# Autodesk Inventor assembly: TR1 Actuator
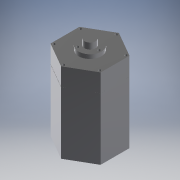
[picture p0: Inventor's stored thumbnail of the model, 180x180]
Saved by Autodesk Inventor 2017 (Build 210142000, 142)
## iProperties
Created: 2018-10-09
Part Number: TR1 Actuator
Document SubType Name: Assembly
Designer: Zach
Author: Zach
## Documents named in this file (15)
- C:\Users\Dell\Documents\GitHub\tr2\Arm Actuator\Arm Actuator.iam
- C:\Users\Dell\Documents\GitHub\tr2\Arm Actuator\TA01.ipt
- C:\Users\Dell\Documents\GitHub\tr2\Arm Actuator\TA02.ipt
- C:\Users\Dell\Documents\GitHub\tr2\Arm Actuator\Arm Actuator\Design Accelerator\Spur Gears2.iam
- C:\Users\Dell\Documents\GitHub\tr2\Arm Actuator\Arm Actuator\Design Accelerator\Spur Gears3.iam
- C:\Users\Dell\Documents\GitHub\tr2\Arm Actuator\EMS22XXX-D28-LSX.ipt
- C:\Users\Dell\Documents\GitHub\tr2\Arm Actuator\12RPM Gear Motor.ipt
- C:\Users\Dell\Documents\GitHub\tr2\Arm Actuator\Slip Ring.ipt
- C:\Users\Dell\Documents\GitHub\tr2\Arm Actuator\TA06.ipt
- C:\Users\Dell\Documents\GitHub\tr2\Arm Actuator\6mm Mounting Hub, thin.ipt
- C:\Users\Dell\Documents\GitHub\tr2\Arm Actuator\Steel Tubing.ipt
- C:\Users\Dell\Documents\GitHub\tr2\Arm Actuator\Flange Bearing.ipt
- C:\Users\Dell\Documents\GitHub\tr2\Arm Actuator\Shaft Collar.ipt
- C:\Users\Dell\Documents\GitHub\tr2\Arm Actuator\Arm Actuator\Design Accelerator\Spur Gear13.ipt
- C:\Users\Dell\Documents\GitHub\tr2\Arm Actuator\6mm Mounting Hub, thick.ipt
## Components (16 placed, 13 different names)
1. TA01:1 — Mate:28, Mate:29, Mate:30
2. TA02:1 — Mate:2, Angle:1, Mate:21, Mate:22, Mate:24, Mate:28, Mate:29, Mate:30, Mate:40, Mate:46, Mate:56, Flush:1, Mate:74, Mate:75, Mate:85, Mate:87, Mate:90, Mate:91
3. TA06:1 — Mate:34, Mate:35, Mate:36, Mate:82, Mate:83
4. Spur Gears:1 [sub-assembly] — Mate:2, Mate:33, Mate:36, Flush:1, Mate:80, Mate:81
5. Spur Gears:4 [sub-assembly] — Mate:23, Mate:24, Mate:54
6. 12RPM Gear Motor:1 — Mate:21, Mate:22, Mate:86, Mate:88, Mate:90, Mate:91
7. EMS22XXX-D28-LSX:1 — Angle:1, Mate:23, Mate:40, Mate:45, Mate:56
8. Slip Ring:1 — Mate:33, Mate:34, Mate:35, Mate:83
9. 6mm Mounting Hub, thin:1 — Mate:45, Mate:46, Mate:54
10. Steel Tubing:1 — Mate:76, Mate:77, Flush:2, Mate:79, Mate:82, Mate:84
11. Flange Bearing:1 — Mate:74, Mate:75, Mate:76, Mate:78
12. Shaft Collar:1 — Mate:77, Mate:78, Flush:2
13. Shaft Collar:2 — Mate:79, Mate:80, Mate:81
14. Flange Bearing:2 — Mate:84, Mate:85
15. Spur Gear1:1 — Mate:88, Mate:89
16. 6mm Mounting Hub, thick:1 — Mate:86, Mate:87, Mate:89
## Relationships (38: Mate 35, Flush 2, Angle 1)
- Mate:2: TA02:1 ↔ Spur Gears:1
- Angle:1 (0 deg): TA02:1 ↔ EMS22XXX-D28-LSX:1
- Mate:21: TA02:1 ↔ 12RPM Gear Motor:1
- Mate:22: TA02:1 ↔ 12RPM Gear Motor:1
- Mate:23: Spur Gears:4 ↔ EMS22XXX-D28-LSX:1
- Mate:24: TA02:1 ↔ Spur Gears:4
- Mate:28: TA01:1 ↔ TA02:1
- Mate:29: TA01:1 ↔ TA02:1
- Mate:30: TA01:1 ↔ TA02:1
- Mate:33: Spur Gears:1 ↔ Slip Ring:1
- Mate:34: TA06:1 ↔ Slip Ring:1
- Mate:35: TA06:1 ↔ Slip Ring:1
- Mate:36: TA06:1 ↔ Spur Gears:1
- Mate:40: TA02:1 ↔ EMS22XXX-D28-LSX:1
- Mate:45: EMS22XXX-D28-LSX:1 ↔ 6mm Mounting Hub, thin:1
- Mate:46: TA02:1 ↔ 6mm Mounting Hub, thin:1
- Mate:54: Spur Gears:4 ↔ 6mm Mounting Hub, thin:1
- Mate:56: TA02:1 ↔ EMS22XXX-D28-LSX:1
- Flush:1: TA02:1 ↔ Spur Gears:1
- Mate:74: TA02:1 ↔ Flange Bearing:1
- Mate:75: TA02:1 ↔ Flange Bearing:1
- Mate:76: Steel Tubing:1 ↔ Flange Bearing:1
- Mate:77: Steel Tubing:1 ↔ Shaft Collar:1
- Mate:78: Flange Bearing:1 ↔ Shaft Collar:1
- Flush:2: Steel Tubing:1 ↔ Shaft Collar:1
- Mate:79: Steel Tubing:1 ↔ Shaft Collar:2
- Mate:80: Spur Gears:1 ↔ Shaft Collar:2
- Mate:81: Spur Gears:1 ↔ Shaft Collar:2
- Mate:82: TA06:1 ↔ Steel Tubing:1
- Mate:83: TA06:1 ↔ Slip Ring:1
- Mate:84: Steel Tubing:1 ↔ Flange Bearing:2
- Mate:85: TA02:1 ↔ Flange Bearing:2
- Mate:86: 12RPM Gear Motor:1 ↔ 6mm Mounting Hub, thick:1
- Mate:87: TA02:1 ↔ 6mm Mounting Hub, thick:1
- Mate:88: 12RPM Gear Motor:1 ↔ Spur Gear1:1
- Mate:89: Spur Gear1:1 ↔ 6mm Mounting Hub, thick:1
- Mate:90: TA02:1 ↔ 12RPM Gear Motor:1
- Mate:91: TA02:1 ↔ 12RPM Gear Motor:1
